# Autodesk Inventor assembly: X Axis
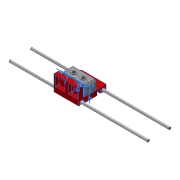
[picture p0: Inventor's stored thumbnail of the model, 180x180]
Saved by Autodesk Inventor 2015 (Build 190159000, 159)
## iProperties
Created: 2020-03-29
Part Number: X Axis
Document SubType Name: Assembly
Designer: Ghassan Yusuf
Author: Ghassan Yusuf
## Documents named in this file (9)
- X:\TAKEONE\Products\takeone-3D-printer\model\3D\X Axis.iam
- X:\TAKEONE\Products\takeone-3D-printer\model\3D\X Axis Shafts.ipt
- X:\TAKEONE\Products\takeone-3D-printer\model\3D\shaft non plane bushes.ipt
- X:\TAKEONE\Products\takeone-3D-printer\model\3D\shaft plane bushes.ipt
- X:\TAKEONE\Products\takeone-3D-printer\model\3D\Carriage nozzel Holder.ipt
- X:\TAKEONE\Products\takeone-3D-printer\model\3D\carriage.ipt
- X:\TAKEONE\Products\takeone-3D-printer\model\3D\betl holder.ipt
- X:\TAKEONE\Products\takeone-3D-printer\model\3D\Extruder Heat Sink.ipt
- X:\TAKEONE\Products\takeone-3D-printer\model\3D\Fan Mounts.ipt
## Components (11 placed, 8 different names)
1. X Axis Shafts:1 — Mate:1, Mate:2, Mate:3, Flush:4, Mate:6
2. shaft non plane bushes:1 — Insert:2, Flush:3, Flush:4
3. shaft plane bushes:2 — Insert:3, Flush:3
4. shaft plane bushes:1 — Insert:4, Flush:2
5. shaft non plane bushes:2 — Insert:1, Flush:2
6. Carriage nozzel Holder:1 — Mate:4, Flush:1, Mate:5, Insert:7, Insert:8, Flush:8
7. carriage:1 — Insert:1, Insert:2, Insert:3, Insert:4, Mate:4, Flush:1, Mate:5, Mate:6, Mate:7, Insert:5, Insert:6, Mate:8, Flush:9
8. betl holder:1 — Mate:7, Insert:5, Insert:6
9. Extruder Heat Sink:1 — Flush:6, Flush:7, Insert:7
10. Extruder Heat Sink:2 — Flush:6, Flush:7, Insert:8
11. Fan Mounts:1 — Mate:8, Flush:8, Flush:9
## Relationships (24: Mate 8, Insert 8, Flush 8)
- Mate:1: X Axis Shafts:1
- Insert:1: shaft non plane bushes:2 ↔ carriage:1
- Insert:2: shaft non plane bushes:1 ↔ carriage:1
- Insert:3: shaft plane bushes:2 ↔ carriage:1
- Insert:4: shaft plane bushes:1 ↔ carriage:1
- Mate:2: X Axis Shafts:1
- Mate:3: X Axis Shafts:1
- Mate:4: Carriage nozzel Holder:1 ↔ carriage:1
- Flush:1: Carriage nozzel Holder:1 ↔ carriage:1
- Mate:5: Carriage nozzel Holder:1 ↔ carriage:1
- Flush:2: shaft plane bushes:1 ↔ shaft non plane bushes:2
- Flush:3: shaft non plane bushes:1 ↔ shaft plane bushes:2
- Flush:4: X Axis Shafts:1 ↔ shaft non plane bushes:1
- Mate:6: X Axis Shafts:1 ↔ carriage:1
- Mate:7: carriage:1 ↔ betl holder:1
- Insert:5: carriage:1 ↔ betl holder:1
- Insert:6: carriage:1 ↔ betl holder:1
- Flush:6: Extruder Heat Sink:1 ↔ Extruder Heat Sink:2
- Flush:7: Extruder Heat Sink:1 ↔ Extruder Heat Sink:2
- Insert:7: Carriage nozzel Holder:1 ↔ Extruder Heat Sink:1
- Insert:8: Carriage nozzel Holder:1 ↔ Extruder Heat Sink:2
- Mate:8: carriage:1 ↔ Fan Mounts:1
- Flush:8: Carriage nozzel Holder:1 ↔ Fan Mounts:1
- Flush:9: carriage:1 ↔ Fan Mounts:1
